# Autodesk Inventor assembly: Assembly_Guinardia_V3
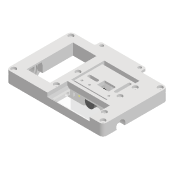
[picture p0: Inventor's stored thumbnail of the model, 180x180]
Saved by Autodesk Inventor 2022 (Build 260153000, 153)
## iProperties
Created: 2022-12-18
Part Number: Assembly_Guinardia_V3
Document SubType Name: Assembly
Designer: diederichbenedict
Author: diederichbenedict
## Documents named in this file (4)
- C:\Users\diederichbenedict\Dropbox\Dokumente\Promotion\PROJECTS\HoLiSheet\INVENTOR\Assembly_Guinardia_V3.iam
- C:\Users\diederichbenedict\Dropbox\Dokumente\Promotion\PROJECTS\HoLiSheet\INVENTOR\Assemlby_Scanner_v1.iam
- C:\Users\diederichbenedict\Dropbox\Dokumente\Promotion\PROJECTS\HoLiSheet\INVENTOR\10_Wellplate_base_v2.ipt
- C:\Users\diederichbenedict\Dropbox\Dokumente\Promotion\PROJECTS\HoLiSheet\INVENTOR\11_Wellplatespacer.ipt
## Components (3 placed, 3 different names)
1. 10_Wellplate_base_v2:1 — Fluchtend:1, Passend:1, Winkel:1, Fluchtend:2, Passend:3, Passend:4, Fluchtend:3, Fluchtend:4, Fluchtend:5
2. Assemlby_Scanner_v1:1 [sub-assembly] — Winkel:1, Fluchtend:2, Passend:3, Passend:4, Fluchtend:3
3. 11_Wellplatespacer:1 — Fluchtend:4, Fluchtend:5
## Relationships (9: Flush 5, Mate 3, Angle 1)
- Fluchtend:1 [Flush]: 10_Wellplate_base_v2:1
- Passend:1 [Mate]: 10_Wellplate_base_v2:1
- Winkel:1 [Angle] (180 deg): 10_Wellplate_base_v2:1 ↔ Assemlby_Scanner_v1:1
- Fluchtend:2 [Flush]: 10_Wellplate_base_v2:1 ↔ Assemlby_Scanner_v1:1
- Passend:3 [Mate]: 10_Wellplate_base_v2:1 ↔ Assemlby_Scanner_v1:1
- Passend:4 [Mate]: 10_Wellplate_base_v2:1 ↔ Assemlby_Scanner_v1:1
- Fluchtend:3 [Flush]: 10_Wellplate_base_v2:1 ↔ Assemlby_Scanner_v1:1
- Fluchtend:4 [Flush]: 10_Wellplate_base_v2:1 ↔ 11_Wellplatespacer:1
- Fluchtend:5 [Flush]: 10_Wellplate_base_v2:1 ↔ 11_Wellplatespacer:1
